(part 1 of 2)
# Autodesk Inventor assembly: mecanum_adaptive_trajectory
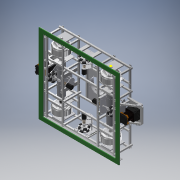
[picture p0: Inventor's stored thumbnail of the model, 180x180]
Saved by Autodesk Inventor 2018 (Build 220112000, 112)
## iProperties
Created: 2018-08-28
Part Number: mecanum_adaptive_trajectory
Material: 一般
Document SubType Name: Assembly
Designer: 澤田　将吾
Mass: 7709.16 g
Surface Area: 29088.3 cm^2
Volume: 5477.44 cm^3
Density: 1.40744 g/cm^3
Author: 澤田　将吾
## Documents named in this file (73)
- C:\Robohan\Svn\2018\自主研究\軌道追従2018\mecanum_adaptive_trajectory.iam
- C:\Robohan\Svn\2018\自主研究\軌道追従2018\既製品\14-KEY-RZ-735.ipt
- C:\Robohan\Svn\2018\自主研究\軌道追従2018\既製品\メカナムホイール.ipt
- C:\Robohan\Svn\2018\自主研究\軌道追従2018\parts\工場工作機\mecanum_wheel_shaft_holder.ipt
- C:\Robohan\Svn\2018\自主研究\軌道追従2018\既製品\mecanum_coupling.ipt
- C:\Robohan\Svn\2018\自主研究\軌道追従2018\parts\センター工作機\motor_plate.ipt
- C:\Robohan\Svn\2018\自主研究\軌道追従2018\parts\センターレーザー\motor-wheel_plate.ipt
- C:\Robohan\Svn\2018\自主研究\軌道追従2018\parts\センター工作機\mecanum_flameA.ipt
- C:\Robohan\Svn\2018\自主研究\軌道追従2018\parts\センター工作機\mecanum_flameB.ipt
- C:\Robohan\Svn\2018\自主研究\軌道追従2018\parts\工場工作機\mecanum_shaft.ipt
- C:\Robohan\Svn\2018\自主研究\軌道追従2018\既製品\14-KEY-RZ-736_MIR.ipt
- C:\Robohan\Svn\2018\自主研究\軌道追従2018\既製品\メカナムホイール_MIR.ipt
- C:\Robohan\Svn\2018\自主研究\軌道追従2018\parts\工場工作機\mecanum_wheel_shaft_holder_MIR.ipt
- C:\Robohan\Svn\2018\自主研究\軌道追従2018\既製品\mecanum_coupling_MIR.ipt
- C:\Robohan\Svn\2018\自主研究\軌道追従2018\parts\センター工作機\motor_plate_MIR.ipt
- C:\Robohan\Svn\2018\自主研究\軌道追従2018\parts\センターレーザー\motor-wheel_plate_MIR.ipt
- C:\Robohan\Svn\2018\自主研究\軌道追従2018\parts\センター工作機\mecanum_flameA_MIR.ipt
- C:\Robohan\Svn\2018\自主研究\軌道追従2018\parts\工場工作機\mecanum_shaft_MIR.ipt
- C:\Robohan\Svn\2018\自主研究\軌道追従2018\parts\センター工作機\mecanum_flameD.ipt
- C:\Robohan\Svn\2018\自主研究\軌道追従2018\parts\センター工作機\mecanum_flameE.ipt
- C:\Robohan\Svn\2018\自主研究\軌道追従2018\既製品\14-KEY-RZ-736_MIR1.ipt
- C:\Robohan\Svn\2018\自主研究\軌道追従2018\既製品\メカナムホイール_MIR1.ipt
- C:\Robohan\Svn\2018\自主研究\軌道追従2018\parts\工場工作機\mecanum_wheel_shaft_holder_MIR1.ipt
- C:\Robohan\Svn\2018\自主研究\軌道追従2018\既製品\mecanum_coupling_MIR1.ipt
- C:\Robohan\Svn\2018\自主研究\軌道追従2018\parts\センター工作機\motor_plate_MIR1.ipt
- C:\Robohan\Svn\2018\自主研究\軌道追従2018\parts\センターレーザー\motor-wheel_plate_MIR1.ipt
- C:\Robohan\Svn\2018\自主研究\軌道追従2018\parts\センター工作機\mecanum_flameA_MIR1.ipt
- C:\Robohan\Svn\2018\自主研究\軌道追従2018\parts\センター工作機\mecanum_flameB_MIR.ipt
- C:\Robohan\Svn\2018\自主研究\軌道追従2018\parts\工場工作機\mecanum_shaft_MIR1.ipt
- C:\Robohan\Svn\2018\自主研究\軌道追従2018\既製品\14-KEY-RZ-736_MIR_MIR.ipt
- C:\Robohan\Svn\2018\自主研究\軌道追従2018\既製品\メカナムホイール_MIR_MIR.ipt
- C:\Robohan\Svn\2018\自主研究\軌道追従2018\parts\工場工作機\mecanum_wheel_shaft_holder_MIR_MIR.ipt
- C:\Robohan\Svn\2018\自主研究\軌道追従2018\既製品\mecanum_coupling_MIR_MIR.ipt
- C:\Robohan\Svn\2018\自主研究\軌道追従2018\parts\センター工作機\motor_plate_MIR_MIR.ipt
- C:\Robohan\Svn\2018\自主研究\軌道追従2018\parts\センターレーザー\motor-wheel_plate_MIR_MIR.ipt
- C:\Robohan\Svn\2018\自主研究\軌道追従2018\parts\センター工作機\mecanum_flameA_MIR_MIR.ipt
- C:\Robohan\Svn\2018\自主研究\軌道追従2018\parts\工場工作機\mecanum_shaft_MIR_MIR.ipt
- C:\Robohan\Svn\2018\自主研究\軌道追従2018\parts\センター工作機\mecanum_flameE_MIR.ipt
- C:\Robohan\Svn\2018\自主研究\軌道追従2018\parts\センター工作機\mecanum_polycaplate.ipt
- C:\Robohan\Svn\2018\自主研究\軌道追従2018\parts\センター工作機\mecanum_polycaplateB.ipt
- C:\Robohan\Svn\2018\自主研究\軌道追従2018\parts\センター工作機\mecanum_polycaplateC.ipt
- C:\Robohan\Svn\2018\自主研究\軌道追従2018\parts\センター工作機\mecanum_angleA.ipt
- C:\Robohan\Svn\2018\自主研究\軌道追従2018\parts\センター工作機\mecanum_angleB.ipt
- C:\Robohan\Svn\2018\自主研究\軌道追従2018\既製品\fan_冶具-01.ipt
- C:\Robohan\Svn\2018\自主研究\軌道追従2018\既製品\bearingA.ipt
- C:\Robohan\Svn\2018\自主研究\軌道追従2018\既製品\mecanum_set_collarA.ipt
- C:\Robohan\Svn\2018\自主研究\軌道追従2018\既製品\Astuto_enc_wheel\Astuto_enc_wheel.iam
- C:\Robohan\Svn\2018\自主研究\軌道追従2018\parts\センター工作機\mecanum_encoder_shaftA.ipt
- C:\Robohan\Svn\2018\自主研究\軌道追従2018\parts\センターレーザー\mecanum_encoder_plateA.ipt
- C:\Robohan\Svn\2018\自主研究\軌道追従2018\parts\センターレーザー\mecanum_encoder_plateB.ipt
- C:\Robohan\Svn\2018\自主研究\軌道追従2018\parts\センター工作機\Astuto_enc_part1.ipt
- C:\Robohan\Svn\2018\自主研究\軌道追従2018\既製品\Astuto_enc_part2.ipt
- C:\Robohan\Svn\2018\自主研究\軌道追従2018\parts\センター工作機\mecanum_encoder_shaftB.ipt
- C:\Robohan\Svn\2018\自主研究\軌道追従2018\既製品\E6A2-CW3C.ipt
- C:\Robohan\Svn\2018\自主研究\軌道追従2018\parts\センターレーザー\mecanum_encoder_plateC.ipt
- C:\Robohan\Svn\2018\自主研究\軌道追従2018\parts\センター工作機\mecanum_encoder_shaftC.ipt
- C:\Robohan\Svn\2018\自主研究\軌道追従2018\parts\センター工作機\Astuto_enc_part3.ipt
- C:\Robohan\Svn\2018\自主研究\軌道追従2018\parts\センターレーザー\mecanum_encoder_plateD.ipt
- C:\Robohan\Svn\2018\自主研究\軌道追従2018\parts\センター工作機\mecanum_encoder_shaftD.ipt
- C:\Robohan\Svn\2018\自主研究\軌道追従2018\既製品\mecanum_encoder_coupling.ipt
- C:\Robohan\Svn\2018\自主研究\軌道追従2018\parts\センター工作機\mecanum_encoder_shaftE.ipt
- C:\Robohan\Svn\2018\自主研究\軌道追従2018\parts\センター工作機\mecanum_encoder_shaftF.ipt
- C:\Robohan\Svn\2018\自主研究\軌道追従2018\既製品\LRF\LRF.iam
- C:\Robohan\Svn\2018\自主研究\軌道追従2018\parts\センター工作機\mecanum_flameF.ipt
- C:\Robohan\Svn\2018\自主研究\軌道追従2018\parts\センター工作機\mecanum_LRF_flameA.ipt
- C:\Robohan\Svn\2018\自主研究\軌道追従2018\parts\センター工作機\mecanum_LRF_plate.ipt
- C:\Robohan\Svn\2018\自主研究\軌道追従2018\parts\センターレーザー\mecanum_gusset_plateA.ipt
- C:\Robohan\Svn\2018\自主研究\軌道追従2018\parts\センター工作機\mecanum_LRF_flameB.ipt
- C:\Robohan\Svn\2018\自主研究\軌道追従2018\parts\センター工作機\mecanum_kusaA.ipt
- C:\Robohan\Svn\2018\自主研究\軌道追従2018\parts\センター工作機\mecanum_kusaB.ipt
- C:\Robohan\Svn\2018\自主研究\軌道追従2018\parts\センター工作機\mecanum_flameG.ipt
- C:\Robohan\Svn\2018\自主研究\軌道追従2018\parts\センター工作機\mecanum_flameH.ipt
- C:\Robohan\Svn\2018\自主研究\軌道追従2018\parts\センターレーザー\mecanum_suction_motor_plate.ipt
## Components (196 placed, 73 different names)
1. 14-KEY-RZ-735:1 — メイト:1, メイト:2, 挿入:8, 挿入:9, 挿入:10, メイト:111
2. メカナムホイール:1 — 挿入:1, 挿入:2, 挿入:3
3. mecanum_wheel_shaft_holder:1 — 挿入:1, 挿入:2, 挿入:3, メイト:4, メイト:9, メイト:10
4. mecanum_coupling:1 — メイト:1, メイト:2, メイト:3, メイト:6, メイト:7, フラッシュ:1
5. motor_plate:1 — 挿入:8, 挿入:9, 挿入:10, メイト:7, 挿入:432, 挿入:433, 挿入:444, 挿入:445
6. motor-wheel_plate:1 — メイト:3, メイト:4, メイト:6, 挿入:4, 挿入:5, 挿入:31, 挿入:32, メイト:42
7. mecanum_flameA:1 — 挿入:4, 挿入:5, 挿入:6, 挿入:7
8. mecanum_flameB:1 — 挿入:6, 挿入:27, 挿入:30, 挿入:63, 挿入:65, 挿入:68, 挿入:71, 挿入:76, 挿入:81, 挿入:211, 挿入:214, 挿入:277, 挿入:278, 挿入:434, 挿入:472
9. mecanum_flameB:2 — 挿入:7, 挿入:28, 挿入:29, 挿入:49, 挿入:53, 挿入:57, 挿入:61, 挿入:75, 挿入:204, 挿入:206, 挿入:212, 挿入:213, 挿入:422, 挿入:424, 挿入:428, 挿入:429, 挿入:430, 挿入:476
10. mecanum_shaft:1 — メイト:9, フラッシュ:1, メイト:10, メイト:41, メイト:43, メイト:111
11. 14-KEY-RZ-736_MIR:1 — メイト:11, メイト:12, 挿入:18, 挿入:19, 挿入:20, メイト:112
12. メカナムホイール_MIR:1 — 挿入:15, 挿入:16, 挿入:17
13. mecanum_wheel_shaft_holder_MIR:1 — 挿入:15, 挿入:16, 挿入:17, メイト:16, メイト:18, メイト:20
14. mecanum_coupling_MIR:1 — メイト:11, メイト:12, メイト:13, メイト:14, メイト:17, メイト:19
15. motor_plate_MIR:1 — メイト:13, 挿入:18, 挿入:19, 挿入:20, 挿入:462, 挿入:463, 挿入:474, 挿入:475
16. motor-wheel_plate_MIR:1 — メイト:14, メイト:16, メイト:17, 挿入:21, 挿入:22, 挿入:40, 挿入:41, メイト:48
17. mecanum_flameA_MIR:1 — 挿入:21, 挿入:22, 挿入:27, 挿入:28
18. mecanum_shaft_MIR:1 — メイト:18, メイト:19, メイト:20, メイト:49, メイト:50, メイト:112
19. mecanum_flameD:1 — 挿入:29, 挿入:30, 挿入:54, 挿入:72, 挿入:153, 挿入:154, 挿入:158, 挿入:159, 挿入:185, 挿入:187, 挿入:190, 挿入:191, 挿入:194, 挿入:238, 挿入:239, 挿入:265, 挿入:266, 挿入:331, 挿入:334
20. mecanum_flameA:2 — 挿入:31, 挿入:32, 挿入:35, 挿入:43
21. mecanum_flameB:3 — 挿入:35, 挿入:42, 挿入:47, 挿入:52, 挿入:56, 挿入:60, 挿入:62, 挿入:78, メイト:67, 挿入:423, 挿入:425, 挿入:443, 挿入:447, 挿入:464, 挿入:465
22. mecanum_flameA_MIR:2 — 挿入:40, 挿入:41, 挿入:42, 挿入:46
23. mecanum_flameB:4 — 挿入:43, 挿入:46, 挿入:48, 挿入:64, 挿入:66, 挿入:69, 挿入:74, 挿入:80, 挿入:84, 挿入:275, 挿入:276, 挿入:446, 挿入:460
24. mecanum_flameD:2 — 挿入:47, 挿入:48, 挿入:55, 挿入:73, 挿入:155, 挿入:156, 挿入:157, 挿入:160, 挿入:186, 挿入:188, 挿入:189, 挿入:192, 挿入:193, 挿入:236, 挿入:237, 挿入:263, 挿入:264, 挿入:332, 挿入:333
25. mecanum_flameE:1 — 挿入:49, 挿入:52, 挿入:181, 挿入:182, 挿入:431, 挿入:442, 挿入:448
26. mecanum_flameE:2 — 挿入:53, 挿入:54, 挿入:55, 挿入:56, 挿入:183, 挿入:184
27. mecanum_flameE:3 — 挿入:57, 挿入:60, 挿入:179, 挿入:180, 挿入:465, 挿入:477
28. mecanum_flameE:4 — 挿入:61, 挿入:62, 挿入:77, 挿入:79, 挿入:177, 挿入:178
29. mecanum_flameE:5 — 挿入:63, 挿入:64, 挿入:68, 挿入:69, 挿入:435, 挿入:449
30. mecanum_flameE:6 — 挿入:65, 挿入:66, 挿入:461, 挿入:473
31. mecanum_flameE:7 — 挿入:71, 挿入:72, 挿入:73, 挿入:74
32. mecanum_flameD:3 — 挿入:75, 挿入:76, 挿入:77, 挿入:82, 挿入:161, 挿入:162, 挿入:165, 挿入:166, 挿入:195, 挿入:198, 挿入:199, 挿入:202, 挿入:249, 挿入:250, 挿入:267, 挿入:268, 挿入:296, 挿入:299
33. mecanum_flameD:4 — 挿入:78, 挿入:79, 挿入:80, 挿入:83, 挿入:163, 挿入:164, 挿入:167, 挿入:168, 挿入:196, 挿入:197, 挿入:200, 挿入:201, 挿入:247, 挿入:248, 挿入:269, 挿入:270, 挿入:297, 挿入:298
34. mecanum_flameE:8 — 挿入:81, 挿入:82, 挿入:83, 挿入:84
35. 14-KEY-RZ-736_MIR1:1 — メイト:22, メイト:23, 挿入:88, 挿入:89, 挿入:90, メイト:113
36. メカナムホイール_MIR1:1 — 挿入:85, 挿入:86, 挿入:87
37. mecanum_wheel_shaft_holder_MIR1:1 — 挿入:85, 挿入:86, 挿入:87, メイト:26, メイト:28, メイト:30
38. mecanum_coupling_MIR1:1 — メイト:22, メイト:23, メイト:24, メイト:25, メイト:27, メイト:29
39. motor_plate_MIR1:1 — メイト:24, 挿入:88, 挿入:89, 挿入:90, 挿入:438, 挿入:439, 挿入:452, 挿入:453
40. motor-wheel_plate_MIR1:1 — メイト:25, メイト:26, メイト:27, 挿入:91, 挿入:92, 挿入:113, 挿入:114, メイト:55
41. mecanum_flameA_MIR1:1 — 挿入:91, 挿入:92, 挿入:93, 挿入:94
42. mecanum_flameB_MIR:1 — 挿入:93, 挿入:106, 挿入:143, 挿入:146, 挿入:148, 挿入:150, 挿入:152, 挿入:153, 挿入:161, 挿入:208, 挿入:210, 挿入:350, 挿入:353, 挿入:437, 挿入:470
43. mecanum_flameB_MIR:2 — 挿入:94, 挿入:105, 挿入:132, 挿入:134, 挿入:138, 挿入:140, 挿入:159, 挿入:162, 挿入:203, 挿入:205, 挿入:207, 挿入:209, 挿入:372, 挿入:374, 挿入:426, 挿入:427, 挿入:440, 挿入:467
44. mecanum_shaft_MIR1:1 — メイト:28, メイト:29, メイト:30, メイト:56, メイト:57, メイト:113
45. 14-KEY-RZ-736_MIR_MIR:1 — メイト:32, メイト:33, 挿入:102, 挿入:103, 挿入:104, メイト:114
46. メカナムホイール_MIR_MIR:1 — 挿入:99, 挿入:100, 挿入:101
47. mecanum_wheel_shaft_holder_MIR_MIR:1 — 挿入:99, 挿入:100, 挿入:101, メイト:36, メイト:39, メイト:40
48. mecanum_coupling_MIR_MIR:1 — メイト:32, メイト:33, メイト:34, メイト:35, メイト:37, フラッシュ:2
49. motor_plate_MIR_MIR:1 — 挿入:102, 挿入:103, 挿入:104, メイト:34, 挿入:458, 挿入:468, 挿入:469
50. motor-wheel_plate_MIR_MIR:1 — メイト:35, メイト:36, メイト:37, 挿入:107, 挿入:108, 挿入:123, 挿入:124, メイト:58
51. mecanum_flameA_MIR_MIR:1 — 挿入:105, 挿入:106, 挿入:107, 挿入:108
52. mecanum_shaft_MIR_MIR:1 — メイト:39, フラッシュ:2, メイト:40, メイト:59, メイト:60, メイト:114
53. mecanum_flameA_MIR1:2 — 挿入:113, 挿入:114, 挿入:118, 挿入:128
54. mecanum_flameB_MIR:3 — 挿入:118, 挿入:122, 挿入:129, 挿入:133, 挿入:135, 挿入:139, 挿入:160, 挿入:164, 挿入:373, 挿入:375, 挿入:454, 挿入:457
55. mecanum_flameA_MIR_MIR:2 — 挿入:122, 挿入:123, 挿入:124, 挿入:125
56. mecanum_flameB_MIR:4 — 挿入:125, 挿入:128, 挿入:142, 挿入:145, 挿入:147, 挿入:149, 挿入:151, 挿入:155, 挿入:163, 挿入:351, 挿入:352, 挿入:450
57. mecanum_flameE_MIR:1 — 挿入:129, 挿入:132, 挿入:173, 挿入:174, 挿入:441, 挿入:455
58. mecanum_flameE_MIR:2 — 挿入:133, 挿入:134, 挿入:157, 挿入:158, 挿入:169, 挿入:170
59. mecanum_flameE_MIR:3 — 挿入:135, 挿入:138, 挿入:175, 挿入:176, 挿入:456, 挿入:466
60. mecanum_flameE_MIR:4 — 挿入:139, 挿入:140, 挿入:166, 挿入:167, 挿入:171, 挿入:172
61. mecanum_flameE_MIR:5 — 挿入:142, 挿入:143, 挿入:145, 挿入:146, 挿入:436, 挿入:451
62. mecanum_flameE_MIR:6 — 挿入:147, 挿入:148, 挿入:459, 挿入:471
63. mecanum_flameE_MIR:7 — 挿入:149, 挿入:150, 挿入:154, 挿入:156
64. mecanum_flameE_MIR:8 — 挿入:151, 挿入:152, 挿入:165, 挿入:168
65. mecanum_polycaplateA:1 — 挿入:169, 挿入:170, 挿入:171, 挿入:172, 挿入:173, 挿入:174, 挿入:175, 挿入:176, 挿入:215, 挿入:216, 挿入:217, 挿入:218
66. mecanum_polycaplate:2 — 挿入:177, 挿入:178, 挿入:179, 挿入:180, 挿入:181, 挿入:182, 挿入:183, 挿入:184, 挿入:219, 挿入:220, 挿入:221, 挿入:222
67. mecanum_polycaplateB:1 — 挿入:185, 挿入:186, 挿入:187, 挿入:188, 挿入:189, 挿入:190, 挿入:191, 挿入:192, 挿入:193, 挿入:194, 挿入:223, 挿入:224, 挿入:225, 挿入:226
68. mecanum_polycaplateB:2 — 挿入:195, 挿入:196, 挿入:197, 挿入:198, 挿入:199, 挿入:200, 挿入:201, 挿入:202, 挿入:227, 挿入:228, 挿入:229, 挿入:230
69. mecanum_polycaplateC:1 — 挿入:203, 挿入:204, 挿入:205, 挿入:206, 挿入:207, 挿入:208, 挿入:209, 挿入:210, 挿入:211, 挿入:212, 挿入:213, 挿入:214
70. mecanum_angleA:1 — 挿入:215, 挿入:216, 挿入:217, 挿入:218, フラッシュ:15, フラッシュ:16, メイト:108
71. mecanum_angleA:2 — 挿入:219, 挿入:220, 挿入:221, 挿入:222, メイト:107, フラッシュ:13, フラッシュ:14
72. mecanum_angleB:1 — 挿入:223, 挿入:224, 挿入:225, 挿入:226, フラッシュ:19, フラッシュ:20, メイト:110
73. mecanum_angleB:2 — 挿入:227, 挿入:228, 挿入:229, 挿入:230, メイト:109, フラッシュ:17, フラッシュ:18
74. fan_冶具-01:1 — 挿入:486, 挿入:487, 挿入:488, 挿入:489, 挿入:490
75. bearingA:1 — メイト:41, メイト:42, 挿入:231
76. mecanum_set_collarA:1 — 挿入:231
77. motor-wheel_plate:2 — メイト:43, 挿入:232, 挿入:233, 挿入:234, 挿入:235, メイト:44, メイト:45
78. motor-wheel_plate:3 — 挿入:232, 挿入:233, 挿入:234, 挿入:235, 挿入:236, 挿入:237, 挿入:238, 挿入:239
79. bearingA:2 — メイト:44, メイト:45, 挿入:240
80. mecanum_set_collarA:2 — 挿入:240
81. bearingA:3 — メイト:48, メイト:49
82. mecanum_set_collarA:3
83. motor-wheel_plate:4
84. motor-wheel_plate:5 — 挿入:247, 挿入:248, 挿入:249, 挿入:250
85. bearingA:4 — メイト:50
86. mecanum_set_collarA:4
87. bearingA:5 — メイト:55
88. mecanum_set_collarA:5 — メイト:56
89. motor-wheel_plate:6
90. motor-wheel_plate:7 — 挿入:263, 挿入:264, 挿入:265, 挿入:266
91. bearingA:6 — メイト:57
92. mecanum_set_collarA:6
93. bearingA:7 — メイト:58, メイト:59
94. mecanum_set_collarA:7
95. motor-wheel_plate:8
96. motor-wheel_plate:9 — 挿入:267, 挿入:268, 挿入:269, 挿入:270
97. bearingA:8 — メイト:60
98. mecanum_set_collarA:8
99. Astuto_enc_wheel:1 [sub-assembly] — メイト:61, メイト:91
100. mecanum_encoder_shaftA:1 — メイト:61, メイト:62, メイト:68, メイト:69, フラッシュ:4, メイト:77
101. mecanum_encoder_plateA:1 — メイト:67, メイト:68, 挿入:281, 挿入:282, フラッシュ:4, メイト:91
102. mecanum_encoder_plateB:1 — メイト:62, 挿入:271, 挿入:272, 挿入:273, 挿入:274, 挿入:280, メイト:70, 挿入:288, 挿入:289, 挿入:290
103. Astuto_enc_part1:2 — メイト:63, メイト:64, 挿入:275, 挿入:278, フラッシュ:3
104. Astuto_enc_part2:2 — メイト:63, メイト:64, 挿入:271, 挿入:272, フラッシュ:3
105. Astuto_enc_part1:3 — 挿入:276, 挿入:277, メイト:66
106. Astuto_enc_part2:3 — 挿入:273, 挿入:274, メイト:66
107. mecanum_encoder_shaftB:1 — 挿入:280, 挿入:281
108. mecanum_encoder_shaftB:2 — 挿入:282
109. E6A2-CW3C:1 — 挿入:283, 挿入:284, メイト:69
110. mecanum_encoder_plateC:1 — 挿入:283, 挿入:284, 挿入:285, 挿入:286, 挿入:287, メイト:78
111. mecanum_encoder_shaftC:1 — 挿入:285, メイト:70, 挿入:289
112. mecanum_encoder_shaftC:2 — 挿入:287, 挿入:290
113. mecanum_encoder_shaftC:3 — 挿入:286, 挿入:288
114. Astuto_enc_wheel:2 [sub-assembly] — メイト:76, メイト:79, メイト:81, メイト:105
115. E6A2-CW3C:2
116. mecanum_encoder_plateC:2 — メイト:80, 挿入:361, 挿入:362, 挿入:363
117. Astuto_enc_part3:1 — 挿入:296, 挿入:297, メイト:72, メイト:74
118. Astuto_enc_part3:2 — 挿入:298, 挿入:299, メイト:73, メイト:75, フラッシュ:6
119. Astuto_enc_part2:4 — メイト:73, メイト:75, 挿入:300, 挿入:303, フラッシュ:6
120. Astuto_enc_part2:5 — メイト:72, メイト:74, 挿入:301, 挿入:302
121. mecanum_encoder_plateD:1 — 挿入:300, 挿入:301, 挿入:302, 挿入:303, メイト:76, 挿入:304, 挿入:305, 挿入:306, フラッシュ:7, メイト:105
122. mecanum_encoder_shaftD:1 — 挿入:304, 挿入:307
123. mecanum_encoder_shaftD:2 — 挿入:305, 挿入:308
124. mecanum_encoder_shaftD:3 — 挿入:306, 挿入:309
125. mecanum_encoder_plateC:3 — 挿入:307, 挿入:308, 挿入:309, 挿入:360, 挿入:364, 挿入:365
126. mecanum_encoder_coupling:1 — メイト:77, メイト:78
127. mecanum_encoder_coupling:2 — メイト:79, メイト:80
128. mecanum_encoder_shaftE:1 — メイト:81, フラッシュ:7
129. Astuto_enc_wheel:3 [sub-assembly] — メイト:106
130. E6A2-CW3C:3
131. mecanum_encoder_plateC:4 — 挿入:355, 挿入:356, 挿入:357
132. Astuto_enc_part3:3 — 挿入:331, 挿入:332
133. Astuto_enc_part3:4 — 挿入:333, 挿入:334
134. Astuto_enc_part2:6
135. Astuto_enc_part2:7
136. mecanum_encoder_plateD:2 — メイト:106
137. mecanum_encoder_shaftD:4
138. mecanum_encoder_shaftD:5
139. mecanum_encoder_shaftD:6
140. mecanum_encoder_plateC:5 — 挿入:354, 挿入:358, 挿入:359
141. mecanum_encoder_coupling:3
142. mecanum_encoder_shaftE:2
143. Astuto_enc_wheel:4 [sub-assembly]
144. mecanum_encoder_shaftA:2
145. mecanum_encoder_plateA:2
146. mecanum_encoder_plateB:2
147. Astuto_enc_part1:4 — 挿入:350, 挿入:351
148. Astuto_enc_part2:8
149. Astuto_enc_part1:5 — 挿入:352, 挿入:353
150. Astuto_enc_part2:9
151. mecanum_encoder_shaftB:3
152. mecanum_encoder_shaftB:4
153. E6A2-CW3C:4
154. mecanum_encoder_plateC:6
155. mecanum_encoder_shaftC:10
156. mecanum_encoder_shaftC:11
157. mecanum_encoder_shaftC:12
158. mecanum_encoder_coupling:4
159. mecanum_encoder_shaftF:1 — 挿入:354, 挿入:355
160. mecanum_encoder_shaftF:2 — 挿入:356, 挿入:358
161. mecanum_encoder_shaftF:3 — 挿入:357, 挿入:359
162. mecanum_encoder_shaftF:4 — 挿入:360, 挿入:361
163. mecanum_encoder_shaftF:5 — 挿入:362, 挿入:364
164. mecanum_encoder_shaftF:6 — 挿入:363, 挿入:365
165. fan_冶具-01:2 — 挿入:491, 挿入:492, 挿入:493, 挿入:494
166. LRF:1 [sub-assembly] — 挿入:384, 挿入:385, 挿入:386, 挿入:387
167. mecanum_flameF:1 — 挿入:372, 挿入:373, 挿入:377, 挿入:394
168. mecanum_flameF:2 — 挿入:374, 挿入:375, 挿入:379, 挿入:401
169. mecanum_LRF_flameA:1 — 挿入:377, 挿入:388, 挿入:389, 挿入:392, 挿入:393, 挿入:427
170. mecanum_LRF_flameA:2 — 挿入:379, 挿入:390, 挿入:391, 挿入:397, 挿入:398, 挿入:426
171. mecanum_LRF_plate:1 — 挿入:384, 挿入:385, 挿入:386, 挿入:387, 挿入:388, 挿入:389, 挿入:390, 挿入:391
172. mecanum_gusset_plateA:1 — 挿入:392, 挿入:393, 挿入:395, 挿入:396
173. mecanum_LRF_flameB:1 — 挿入:394, 挿入:395, 挿入:396
174. mecanum_gusset_plateA:2 — 挿入:397, 挿入:398, 挿入:399, 挿入:400
175. mecanum_LRF_flameB:2 — 挿入:399, 挿入:400, 挿入:401
176. LRF:3 [sub-assembly]
177. mecanum_flameF:3 — 挿入:422, 挿入:423
178. mecanum_flameF:4 — 挿入:424, 挿入:425
179. mecanum_LRF_flameA:3 — 挿入:428
180. mecanum_LRF_flameA:4 — 挿入:429
181. mecanum_LRF_plate:2
182. mecanum_gusset_plateA:3
183. mecanum_LRF_flameB:3
184. mecanum_gusset_plateA:4
185. mecanum_LRF_flameB:4
186. mecanum_kusaA:1 — フラッシュ:15, フラッシュ:16, メイト:108
187. mecanum_kusaA:2 — メイト:107, フラッシュ:13, フラッシュ:14
188. mecanum_kusaB:1 — メイト:109, フラッシュ:17, フラッシュ:18
189. mecanum_kusaB:2 — フラッシュ:19, フラッシュ:20, メイト:110
190. mecanum_flameG:1 — 挿入:430, 挿入:431, 挿入:432, 挿入:433, 挿入:434, 挿入:435, 挿入:436, 挿入:437, 挿入:438, 挿入:439, 挿入:440, 挿入:441, 挿入:479, 挿入:481
191. mecanum_flameG:2 — 挿入:442, 挿入:443, 挿入:444, 挿入:445, 挿入:446, 挿入:447, 挿入:448, 挿入:449, 挿入:450, 挿入:451, 挿入:452, 挿入:453, 挿入:454, 挿入:455
192. mecanum_flameG:3 — 挿入:456, 挿入:457, 挿入:458, 挿入:459, 挿入:460, 挿入:461, 挿入:462, 挿入:463, 挿入:464
193. mecanum_flameG:4 — 挿入:466, 挿入:467, 挿入:468, 挿入:469, 挿入:470, 挿入:471, 挿入:472, 挿入:473, 挿入:474, 挿入:475, 挿入:476, 挿入:477, 挿入:478, 挿入:480
194. mecanum_flameH:1 — 挿入:478, 挿入:479, 挿入:482, 挿入:484
195. mecanum_suction_motor_plate:1 — 挿入:482, 挿入:483, 挿入:484, 挿入:485, 挿入:486, 挿入:487, 挿入:488, 挿入:489, 挿入:490, 挿入:491, 挿入:492, 挿入:493, 挿入:494
196. mecanum_flameH:2 — 挿入:480, 挿入:481, 挿入:483, 挿入:485
## Relationships (548: Insert 425, Mate 105, Flush 18)
- 挿入:1 [Insert]: メカナムホイール:1 ↔ mecanum_wheel_shaft_holder:1
- 挿入:2 [Insert]: メカナムホイール:1 ↔ mecanum_wheel_shaft_holder:1
- 挿入:3 [Insert]: メカナムホイール:1 ↔ mecanum_wheel_shaft_holder:1
- メイト:1 [Mate]: 14-KEY-RZ-735:1 ↔ mecanum_coupling:1
- メイト:2 [Mate] (3 mm): 14-KEY-RZ-735:1 ↔ mecanum_coupling:1
- メイト:3 [Mate]: mecanum_coupling:1 ↔ motor-wheel_plate:1
- メイト:4 [Mate]: mecanum_wheel_shaft_holder:1 ↔ motor-wheel_plate:1
- メイト:6 [Mate] (5 mm): mecanum_coupling:1 ↔ motor-wheel_plate:1
- 挿入:4 [Insert]: motor-wheel_plate:1 ↔ mecanum_flameA:1
- 挿入:5 [Insert]: motor-wheel_plate:1 ↔ mecanum_flameA:1
- 挿入:6 [Insert]: mecanum_flameA:1 ↔ mecanum_flameB:1
- 挿入:7 [Insert]: mecanum_flameA:1 ↔ mecanum_flameB:2
- 挿入:8 [Insert]: 14-KEY-RZ-735:1 ↔ motor_plate:1
- 挿入:9 [Insert]: 14-KEY-RZ-735:1 ↔ motor_plate:1
- 挿入:10 [Insert]: 14-KEY-RZ-735:1 ↔ motor_plate:1
- メイト:7 [Mate] (5 mm): mecanum_coupling:1 ↔ motor_plate:1
- メイト:9 [Mate]: mecanum_wheel_shaft_holder:1 ↔ mecanum_shaft:1
- フラッシュ:1 [Flush]: mecanum_coupling:1 ↔ mecanum_shaft:1
- メイト:10 [Mate]: mecanum_wheel_shaft_holder:1 ↔ mecanum_shaft:1
- 挿入:15 [Insert]: メカナムホイール_MIR:1 ↔ mecanum_wheel_shaft_holder_MIR:1
- 挿入:16 [Insert]: メカナムホイール_MIR:1 ↔ mecanum_wheel_shaft_holder_MIR:1
- 挿入:17 [Insert]: メカナムホイール_MIR:1 ↔ mecanum_wheel_shaft_holder_MIR:1
- メイト:11 [Mate] (3 mm): 14-KEY-RZ-736_MIR:1 ↔ mecanum_coupling_MIR:1
- メイト:12 [Mate]: 14-KEY-RZ-736_MIR:1 ↔ mecanum_coupling_MIR:1
- メイト:13 [Mate] (5 mm): mecanum_coupling_MIR:1 ↔ motor_plate_MIR:1
- 挿入:18 [Insert]: 14-KEY-RZ-736_MIR:1 ↔ motor_plate_MIR:1
- 挿入:19 [Insert]: 14-KEY-RZ-736_MIR:1 ↔ motor_plate_MIR:1
- 挿入:20 [Insert]: 14-KEY-RZ-736_MIR:1 ↔ motor_plate_MIR:1
- メイト:14 [Mate] (5 mm): mecanum_coupling_MIR:1 ↔ motor-wheel_plate_MIR:1
- メイト:16 [Mate]: mecanum_wheel_shaft_holder_MIR:1 ↔ motor-wheel_plate_MIR:1
- メイト:17 [Mate]: mecanum_coupling_MIR:1 ↔ motor-wheel_plate_MIR:1
- 挿入:21 [Insert]: motor-wheel_plate_MIR:1 ↔ mecanum_flameA_MIR:1
- 挿入:22 [Insert]: motor-wheel_plate_MIR:1 ↔ mecanum_flameA_MIR:1
- メイト:18 [Mate]: mecanum_wheel_shaft_holder_MIR:1 ↔ mecanum_shaft_MIR:1
- メイト:19 [Mate]: mecanum_coupling_MIR:1 ↔ mecanum_shaft_MIR:1
- メイト:20 [Mate]: mecanum_wheel_shaft_holder_MIR:1 ↔ mecanum_shaft_MIR:1
- 挿入:27 [Insert]: mecanum_flameB:1 ↔ mecanum_flameA_MIR:1
- 挿入:28 [Insert]: mecanum_flameB:2 ↔ mecanum_flameA_MIR:1
- 挿入:29 [Insert]: mecanum_flameB:2 ↔ mecanum_flameD:1
- 挿入:30 [Insert]: mecanum_flameB:1 ↔ mecanum_flameD:1
- 挿入:31 [Insert]: motor-wheel_plate:1 ↔ mecanum_flameA:2
- 挿入:32 [Insert]: motor-wheel_plate:1 ↔ mecanum_flameA:2
- 挿入:35 [Insert]: mecanum_flameA:2 ↔ mecanum_flameB:3
- 挿入:40 [Insert]: motor-wheel_plate_MIR:1 ↔ mecanum_flameA_MIR:2
- 挿入:41 [Insert]: motor-wheel_plate_MIR:1 ↔ mecanum_flameA_MIR:2
- 挿入:42 [Insert]: mecanum_flameB:3 ↔ mecanum_flameA_MIR:2
- 挿入:43 [Insert]: mecanum_flameA:2 ↔ mecanum_flameB:4
- 挿入:46 [Insert]: mecanum_flameA_MIR:2 ↔ mecanum_flameB:4
- 挿入:47 [Insert]: mecanum_flameB:3 ↔ mecanum_flameD:2
- 挿入:48 [Insert]: mecanum_flameB:4 ↔ mecanum_flameD:2
- 挿入:49 [Insert]: mecanum_flameB:2 ↔ mecanum_flameE:1
- 挿入:52 [Insert]: mecanum_flameB:3 ↔ mecanum_flameE:1
- 挿入:53 [Insert]: mecanum_flameB:2 ↔ mecanum_flameE:2
- 挿入:54 [Insert]: mecanum_flameD:1 ↔ mecanum_flameE:2
- 挿入:55 [Insert]: mecanum_flameD:2 ↔ mecanum_flameE:2
- 挿入:56 [Insert]: mecanum_flameB:3 ↔ mecanum_flameE:2
- 挿入:57 [Insert]: mecanum_flameB:2 ↔ mecanum_flameE:3
- 挿入:60 [Insert]: mecanum_flameB:3 ↔ mecanum_flameE:3
- 挿入:61 [Insert]: mecanum_flameB:2 ↔ mecanum_flameE:4
- 挿入:62 [Insert]: mecanum_flameB:3 ↔ mecanum_flameE:4
- 挿入:63 [Insert]: mecanum_flameB:1 ↔ mecanum_flameE:5
- 挿入:64 [Insert]: mecanum_flameB:4 ↔ mecanum_flameE:5
- 挿入:65 [Insert]: mecanum_flameB:1 ↔ mecanum_flameE:6
- 挿入:66 [Insert]: mecanum_flameB:4 ↔ mecanum_flameE:6
- 挿入:68 [Insert]: mecanum_flameB:1 ↔ mecanum_flameE:5
- 挿入:69 [Insert]: mecanum_flameB:4 ↔ mecanum_flameE:5
- 挿入:71 [Insert]: mecanum_flameB:1 ↔ mecanum_flameE:7
- 挿入:72 [Insert]: mecanum_flameD:1 ↔ mecanum_flameE:7
- 挿入:73 [Insert]: mecanum_flameD:2 ↔ mecanum_flameE:7
- 挿入:74 [Insert]: mecanum_flameB:4 ↔ mecanum_flameE:7
- 挿入:75 [Insert]: mecanum_flameB:2 ↔ mecanum_flameD:3
- 挿入:76 [Insert]: mecanum_flameB:1 ↔ mecanum_flameD:3
- 挿入:77 [Insert]: mecanum_flameE:4 ↔ mecanum_flameD:3
- 挿入:78 [Insert]: mecanum_flameB:3 ↔ mecanum_flameD:4
- 挿入:79 [Insert]: mecanum_flameE:4 ↔ mecanum_flameD:4
- 挿入:80 [Insert]: mecanum_flameB:4 ↔ mecanum_flameD:4
- 挿入:81 [Insert]: mecanum_flameB:1 ↔ mecanum_flameE:8
- 挿入:82 [Insert]: mecanum_flameD:3 ↔ mecanum_flameE:8
- 挿入:83 [Insert]: mecanum_flameD:4 ↔ mecanum_flameE:8
- 挿入:84 [Insert]: mecanum_flameB:4 ↔ mecanum_flameE:8
- 挿入:85 [Insert]: メカナムホイール_MIR1:1 ↔ mecanum_wheel_shaft_holder_MIR1:1
- 挿入:86 [Insert]: メカナムホイール_MIR1:1 ↔ mecanum_wheel_shaft_holder_MIR1:1
- 挿入:87 [Insert]: メカナムホイール_MIR1:1 ↔ mecanum_wheel_shaft_holder_MIR1:1
- メイト:22 [Mate] (3 mm): 14-KEY-RZ-736_MIR1:1 ↔ mecanum_coupling_MIR1:1
- メイト:23 [Mate]: 14-KEY-RZ-736_MIR1:1 ↔ mecanum_coupling_MIR1:1
- メイト:24 [Mate] (5 mm): mecanum_coupling_MIR1:1 ↔ motor_plate_MIR1:1
- 挿入:88 [Insert]: 14-KEY-RZ-736_MIR1:1 ↔ motor_plate_MIR1:1
- 挿入:89 [Insert]: 14-KEY-RZ-736_MIR1:1 ↔ motor_plate_MIR1:1
- 挿入:90 [Insert]: 14-KEY-RZ-736_MIR1:1 ↔ motor_plate_MIR1:1
- メイト:25 [Mate] (5 mm): mecanum_coupling_MIR1:1 ↔ motor-wheel_plate_MIR1:1
- メイト:26 [Mate]: mecanum_wheel_shaft_holder_MIR1:1 ↔ motor-wheel_plate_MIR1:1
- メイト:27 [Mate]: mecanum_coupling_MIR1:1 ↔ motor-wheel_plate_MIR1:1
- 挿入:91 [Insert]: motor-wheel_plate_MIR1:1 ↔ mecanum_flameA_MIR1:1
- 挿入:92 [Insert]: motor-wheel_plate_MIR1:1 ↔ mecanum_flameA_MIR1:1
- 挿入:93 [Insert]: mecanum_flameA_MIR1:1 ↔ mecanum_flameB_MIR:1
- 挿入:94 [Insert]: mecanum_flameA_MIR1:1 ↔ mecanum_flameB_MIR:2
- メイト:28 [Mate]: mecanum_wheel_shaft_holder_MIR1:1 ↔ mecanum_shaft_MIR1:1
- メイト:29 [Mate]: mecanum_coupling_MIR1:1 ↔ mecanum_shaft_MIR1:1
- メイト:30 [Mate]: mecanum_wheel_shaft_holder_MIR1:1 ↔ mecanum_shaft_MIR1:1
- 挿入:99 [Insert]: メカナムホイール_MIR_MIR:1 ↔ mecanum_wheel_shaft_holder_MIR_MIR:1
- 挿入:100 [Insert]: メカナムホイール_MIR_MIR:1 ↔ mecanum_wheel_shaft_holder_MIR_MIR:1
- 挿入:101 [Insert]: メカナムホイール_MIR_MIR:1 ↔ mecanum_wheel_shaft_holder_MIR_MIR:1
- メイト:32 [Mate]: 14-KEY-RZ-736_MIR_MIR:1 ↔ mecanum_coupling_MIR_MIR:1
- メイト:33 [Mate] (3 mm): 14-KEY-RZ-736_MIR_MIR:1 ↔ mecanum_coupling_MIR_MIR:1
- 挿入:102 [Insert]: 14-KEY-RZ-736_MIR_MIR:1 ↔ motor_plate_MIR_MIR:1
- 挿入:103 [Insert]: 14-KEY-RZ-736_MIR_MIR:1 ↔ motor_plate_MIR_MIR:1
- 挿入:104 [Insert]: 14-KEY-RZ-736_MIR_MIR:1 ↔ motor_plate_MIR_MIR:1
- メイト:34 [Mate] (5 mm): mecanum_coupling_MIR_MIR:1 ↔ motor_plate_MIR_MIR:1
- メイト:35 [Mate]: mecanum_coupling_MIR_MIR:1 ↔ motor-wheel_plate_MIR_MIR:1
- メイト:36 [Mate]: mecanum_wheel_shaft_holder_MIR_MIR:1 ↔ motor-wheel_plate_MIR_MIR:1
- メイト:37 [Mate] (5 mm): mecanum_coupling_MIR_MIR:1 ↔ motor-wheel_plate_MIR_MIR:1
- 挿入:105 [Insert]: mecanum_flameB_MIR:2 ↔ mecanum_flameA_MIR_MIR:1
- 挿入:106 [Insert]: mecanum_flameB_MIR:1 ↔ mecanum_flameA_MIR_MIR:1
- 挿入:107 [Insert]: motor-wheel_plate_MIR_MIR:1 ↔ mecanum_flameA_MIR_MIR:1
- 挿入:108 [Insert]: motor-wheel_plate_MIR_MIR:1 ↔ mecanum_flameA_MIR_MIR:1
- メイト:39 [Mate]: mecanum_wheel_shaft_holder_MIR_MIR:1 ↔ mecanum_shaft_MIR_MIR:1
- フラッシュ:2 [Flush]: mecanum_coupling_MIR_MIR:1 ↔ mecanum_shaft_MIR_MIR:1
- メイト:40 [Mate]: mecanum_wheel_shaft_holder_MIR_MIR:1 ↔ mecanum_shaft_MIR_MIR:1
- 挿入:113 [Insert]: motor-wheel_plate_MIR1:1 ↔ mecanum_flameA_MIR1:2
- 挿入:114 [Insert]: motor-wheel_plate_MIR1:1 ↔ mecanum_flameA_MIR1:2
- 挿入:118 [Insert]: mecanum_flameA_MIR1:2 ↔ mecanum_flameB_MIR:3
- 挿入:122 [Insert]: mecanum_flameB_MIR:3 ↔ mecanum_flameA_MIR_MIR:2
- 挿入:123 [Insert]: motor-wheel_plate_MIR_MIR:1 ↔ mecanum_flameA_MIR_MIR:2
- 挿入:124 [Insert]: motor-wheel_plate_MIR_MIR:1 ↔ mecanum_flameA_MIR_MIR:2
- 挿入:125 [Insert]: mecanum_flameA_MIR_MIR:2 ↔ mecanum_flameB_MIR:4
- 挿入:128 [Insert]: mecanum_flameA_MIR1:2 ↔ mecanum_flameB_MIR:4
- 挿入:129 [Insert]: mecanum_flameB_MIR:3 ↔ mecanum_flameE_MIR:1
- 挿入:132 [Insert]: mecanum_flameB_MIR:2 ↔ mecanum_flameE_MIR:1
- 挿入:133 [Insert]: mecanum_flameB_MIR:3 ↔ mecanum_flameE_MIR:2
- 挿入:134 [Insert]: mecanum_flameB_MIR:2 ↔ mecanum_flameE_MIR:2
- 挿入:135 [Insert]: mecanum_flameB_MIR:3 ↔ mecanum_flameE_MIR:3
- 挿入:138 [Insert]: mecanum_flameB_MIR:2 ↔ mecanum_flameE_MIR:3
- 挿入:139 [Insert]: mecanum_flameB_MIR:3 ↔ mecanum_flameE_MIR:4
- 挿入:140 [Insert]: mecanum_flameB_MIR:2 ↔ mecanum_flameE_MIR:4
- 挿入:142 [Insert]: mecanum_flameB_MIR:4 ↔ mecanum_flameE_MIR:5
- 挿入:143 [Insert]: mecanum_flameB_MIR:1 ↔ mecanum_flameE_MIR:5
- 挿入:145 [Insert]: mecanum_flameB_MIR:4 ↔ mecanum_flameE_MIR:5
- 挿入:146 [Insert]: mecanum_flameB_MIR:1 ↔ mecanum_flameE_MIR:5
- 挿入:147 [Insert]: mecanum_flameB_MIR:4 ↔ mecanum_flameE_MIR:6
- 挿入:148 [Insert]: mecanum_flameB_MIR:1 ↔ mecanum_flameE_MIR:6
- 挿入:149 [Insert]: mecanum_flameB_MIR:4 ↔ mecanum_flameE_MIR:7
- 挿入:150 [Insert]: mecanum_flameB_MIR:1 ↔ mecanum_flameE_MIR:7
- 挿入:151 [Insert]: mecanum_flameB_MIR:4 ↔ mecanum_flameE_MIR:8
- 挿入:152 [Insert]: mecanum_flameB_MIR:1 ↔ mecanum_flameE_MIR:8
- 挿入:153 [Insert]: mecanum_flameD:1 ↔ mecanum_flameB_MIR:1
- 挿入:154 [Insert]: mecanum_flameD:1 ↔ mecanum_flameE_MIR:7
- 挿入:155 [Insert]: mecanum_flameD:2 ↔ mecanum_flameB_MIR:4
- 挿入:156 [Insert]: mecanum_flameD:2 ↔ mecanum_flameE_MIR:7
- 挿入:157 [Insert]: mecanum_flameD:2 ↔ mecanum_flameE_MIR:2
- 挿入:158 [Insert]: mecanum_flameD:1 ↔ mecanum_flameE_MIR:2
- 挿入:159 [Insert]: mecanum_flameD:1 ↔ mecanum_flameB_MIR:2
- 挿入:160 [Insert]: mecanum_flameD:2 ↔ mecanum_flameB_MIR:3
- 挿入:161 [Insert]: mecanum_flameD:3 ↔ mecanum_flameB_MIR:1
- 挿入:162 [Insert]: mecanum_flameD:3 ↔ mecanum_flameB_MIR:2
- 挿入:163 [Insert]: mecanum_flameD:4 ↔ mecanum_flameB_MIR:4
- 挿入:164 [Insert]: mecanum_flameD:4 ↔ mecanum_flameB_MIR:3
- 挿入:165 [Insert]: mecanum_flameD:3 ↔ mecanum_flameE_MIR:8
- 挿入:166 [Insert]: mecanum_flameD:3 ↔ mecanum_flameE_MIR:4
- 挿入:167 [Insert]: mecanum_flameD:4 ↔ mecanum_flameE_MIR:4
- 挿入:168 [Insert]: mecanum_flameD:4 ↔ mecanum_flameE_MIR:8
- 挿入:169 [Insert]: mecanum_flameE_MIR:2 ↔ mecanum_polycaplateA:1
- 挿入:170 [Insert]: mecanum_flameE_MIR:2 ↔ mecanum_polycaplateA:1
- 挿入:171 [Insert]: mecanum_flameE_MIR:4 ↔ mecanum_polycaplateA:1
- 挿入:172 [Insert]: mecanum_flameE_MIR:4 ↔ mecanum_polycaplateA:1
- 挿入:173 [Insert]: mecanum_flameE_MIR:1 ↔ mecanum_polycaplateA:1
- 挿入:174 [Insert]: mecanum_flameE_MIR:1 ↔ mecanum_polycaplateA:1
- 挿入:175 [Insert]: mecanum_flameE_MIR:3 ↔ mecanum_polycaplateA:1
- 挿入:176 [Insert]: mecanum_flameE_MIR:3 ↔ mecanum_polycaplateA:1
- 挿入:177 [Insert]: mecanum_flameE:4 ↔ mecanum_polycaplate:2
- 挿入:178 [Insert]: mecanum_flameE:4 ↔ mecanum_polycaplate:2
- 挿入:179 [Insert]: mecanum_flameE:3 ↔ mecanum_polycaplate:2
- 挿入:180 [Insert]: mecanum_flameE:3 ↔ mecanum_polycaplate:2
- 挿入:181 [Insert]: mecanum_flameE:1 ↔ mecanum_polycaplate:2
- 挿入:182 [Insert]: mecanum_flameE:1 ↔ mecanum_polycaplate:2
- 挿入:183 [Insert]: mecanum_flameE:2 ↔ mecanum_polycaplate:2
- 挿入:184 [Insert]: mecanum_flameE:2 ↔ mecanum_polycaplate:2
- 挿入:185 [Insert]: mecanum_flameD:1 ↔ mecanum_polycaplateB:1
- 挿入:186 [Insert]: mecanum_flameD:2 ↔ mecanum_polycaplateB:1
- 挿入:187 [Insert]: mecanum_flameD:1 ↔ mecanum_polycaplateB:1
- 挿入:188 [Insert]: mecanum_flameD:2 ↔ mecanum_polycaplateB:1
- 挿入:189 [Insert]: mecanum_flameD:2 ↔ mecanum_polycaplateB:1
- 挿入:190 [Insert]: mecanum_flameD:1 ↔ mecanum_polycaplateB:1
- 挿入:191 [Insert]: mecanum_flameD:1 ↔ mecanum_polycaplateB:1
- 挿入:192 [Insert]: mecanum_flameD:2 ↔ mecanum_polycaplateB:1
- 挿入:193 [Insert]: mecanum_flameD:2 ↔ mecanum_polycaplateB:1
- 挿入:194 [Insert]: mecanum_flameD:1 ↔ mecanum_polycaplateB:1
- 挿入:195 [Insert]: mecanum_flameD:3 ↔ mecanum_polycaplateB:2
- 挿入:196 [Insert]: mecanum_flameD:4 ↔ mecanum_polycaplateB:2
- 挿入:197 [Insert]: mecanum_flameD:4 ↔ mecanum_polycaplateB:2
- 挿入:198 [Insert]: mecanum_flameD:3 ↔ mecanum_polycaplateB:2
- 挿入:199 [Insert]: mecanum_flameD:3 ↔ mecanum_polycaplateB:2
- 挿入:200 [Insert]: mecanum_flameD:4 ↔ mecanum_polycaplateB:2
- 挿入:201 [Insert]: mecanum_flameD:4 ↔ mecanum_polycaplateB:2
- 挿入:202 [Insert]: mecanum_flameD:3 ↔ mecanum_polycaplateB:2
- 挿入:203 [Insert]: mecanum_flameB_MIR:2 ↔ mecanum_polycaplateC:1
- 挿入:204 [Insert]: mecanum_flameB:2 ↔ mecanum_polycaplateC:1
- 挿入:205 [Insert]: mecanum_flameB_MIR:2 ↔ mecanum_polycaplateC:1
- 挿入:206 [Insert]: mecanum_flameB:2 ↔ mecanum_polycaplateC:1
- 挿入:207 [Insert]: mecanum_flameB_MIR:2 ↔ mecanum_polycaplateC:1
- 挿入:208 [Insert]: mecanum_flameB_MIR:1 ↔ mecanum_polycaplateC:1
- 挿入:209 [Insert]: mecanum_flameB_MIR:2 ↔ mecanum_polycaplateC:1
- 挿入:210 [Insert]: mecanum_flameB_MIR:1 ↔ mecanum_polycaplateC:1
- 挿入:211 [Insert]: mecanum_flameB:1 ↔ mecanum_polycaplateC:1
- 挿入:212 [Insert]: mecanum_flameB:2 ↔ mecanum_polycaplateC:1
- 挿入:213 [Insert]: mecanum_flameB:2 ↔ mecanum_polycaplateC:1
- 挿入:214 [Insert]: mecanum_flameB:1 ↔ mecanum_polycaplateC:1
- 挿入:215 [Insert]: mecanum_polycaplateA:1 ↔ mecanum_angleA:1
- 挿入:216 [Insert]: mecanum_polycaplateA:1 ↔ mecanum_angleA:1
- 挿入:217 [Insert]: mecanum_polycaplateA:1 ↔ mecanum_angleA:1
- 挿入:218 [Insert]: mecanum_polycaplateA:1 ↔ mecanum_angleA:1
- 挿入:219 [Insert]: mecanum_polycaplate:2 ↔ mecanum_angleA:2
- 挿入:220 [Insert]: mecanum_polycaplate:2 ↔ mecanum_angleA:2
- 挿入:221 [Insert]: mecanum_polycaplate:2 ↔ mecanum_angleA:2
- 挿入:222 [Insert]: mecanum_polycaplate:2 ↔ mecanum_angleA:2
- 挿入:223 [Insert]: mecanum_polycaplateB:1 ↔ mecanum_angleB:1
- 挿入:224 [Insert]: mecanum_polycaplateB:1 ↔ mecanum_angleB:1
- 挿入:225 [Insert]: mecanum_polycaplateB:1 ↔ mecanum_angleB:1
- 挿入:226 [Insert]: mecanum_polycaplateB:1 ↔ mecanum_angleB:1
- 挿入:227 [Insert]: mecanum_polycaplateB:2 ↔ mecanum_angleB:2
- 挿入:228 [Insert]: mecanum_polycaplateB:2 ↔ mecanum_angleB:2
- 挿入:229 [Insert]: mecanum_polycaplateB:2 ↔ mecanum_angleB:2
- 挿入:230 [Insert]: mecanum_polycaplateB:2 ↔ mecanum_angleB:2
- メイト:41 [Mate]: mecanum_shaft:1 ↔ bearingA:1
- メイト:42 [Mate]: motor-wheel_plate:1 ↔ bearingA:1
- 挿入:231 [Insert]: bearingA:1 ↔ mecanum_set_collarA:1
- メイト:43 [Mate]: mecanum_shaft:1 ↔ motor-wheel_plate:2
- 挿入:232 [Insert]: motor-wheel_plate:2 ↔ motor-wheel_plate:3
- 挿入:233 [Insert]: motor-wheel_plate:2 ↔ motor-wheel_plate:3
- 挿入:234 [Insert]: motor-wheel_plate:2 ↔ motor-wheel_plate:3
- 挿入:235 [Insert]: motor-wheel_plate:2 ↔ motor-wheel_plate:3
- 挿入:236 [Insert]: mecanum_flameD:2 ↔ motor-wheel_plate:3
- 挿入:237 [Insert]: mecanum_flameD:2 ↔ motor-wheel_plate:3
- 挿入:238 [Insert]: mecanum_flameD:1 ↔ motor-wheel_plate:3
- 挿入:239 [Insert]: mecanum_flameD:1 ↔ motor-wheel_plate:3
- メイト:44 [Mate]: motor-wheel_plate:2 ↔ bearingA:2
- メイト:45 [Mate]: motor-wheel_plate:2 ↔ bearingA:2
- 挿入:240 [Insert]: bearingA:2 ↔ mecanum_set_collarA:2
- [Insert]: bearingA:3 ↔ mecanum_set_collarA:3
- [Insert]: motor-wheel_plate:4 ↔ motor-wheel_plate:5
- [Insert]: motor-wheel_plate:4 ↔ motor-wheel_plate:5
- [Insert]: motor-wheel_plate:4 ↔ motor-wheel_plate:5
- [Insert]: motor-wheel_plate:4 ↔ motor-wheel_plate:5
- [Mate]: motor-wheel_plate:4 ↔ bearingA:4
- [Mate]: motor-wheel_plate:4 ↔ bearingA:4
- [Insert]: bearingA:4 ↔ mecanum_set_collarA:4
- メイト:48 [Mate]: motor-wheel_plate_MIR:1 ↔ bearingA:3
- メイト:49 [Mate]: mecanum_shaft_MIR:1 ↔ bearingA:3
- メイト:50 [Mate]: mecanum_shaft_MIR:1 ↔ bearingA:4
- 挿入:247 [Insert]: mecanum_flameD:4 ↔ motor-wheel_plate:5
- 挿入:248 [Insert]: mecanum_flameD:4 ↔ motor-wheel_plate:5
- 挿入:249 [Insert]: mecanum_flameD:3 ↔ motor-wheel_plate:5
- 挿入:250 [Insert]: mecanum_flameD:3 ↔ motor-wheel_plate:5
- [Insert]: bearingA:5 ↔ mecanum_set_collarA:5
- [Insert]: motor-wheel_plate:6 ↔ motor-wheel_plate:7
- [Insert]: motor-wheel_plate:6 ↔ motor-wheel_plate:7
- [Insert]: motor-wheel_plate:6 ↔ motor-wheel_plate:7
- [Insert]: motor-wheel_plate:6 ↔ motor-wheel_plate:7
- [Mate]: motor-wheel_plate:6 ↔ bearingA:6
- [Mate]: motor-wheel_plate:6 ↔ bearingA:6
- [Insert]: bearingA:6 ↔ mecanum_set_collarA:6
- [Insert]: bearingA:7 ↔ mecanum_set_collarA:7
- [Insert]: motor-wheel_plate:8 ↔ motor-wheel_plate:9
- [Insert]: motor-wheel_plate:8 ↔ motor-wheel_plate:9
- [Insert]: motor-wheel_plate:8 ↔ motor-wheel_plate:9
- [Insert]: motor-wheel_plate:8 ↔ motor-wheel_plate:9
- [Mate]: motor-wheel_plate:8 ↔ bearingA:8
- [Mate]: motor-wheel_plate:8 ↔ bearingA:8
- [Insert]: bearingA:8 ↔ mecanum_set_collarA:8
- メイト:55 [Mate]: motor-wheel_plate_MIR1:1 ↔ bearingA:5
- メイト:56 [Mate]: mecanum_shaft_MIR1:1 ↔ mecanum_set_collarA:5
- メイト:57 [Mate]: mecanum_shaft_MIR1:1 ↔ bearingA:6
- 挿入:263 [Insert]: mecanum_flameD:2 ↔ motor-wheel_plate:7
- 挿入:264 [Insert]: mecanum_flameD:2 ↔ motor-wheel_plate:7
- 挿入:265 [Insert]: mecanum_flameD:1 ↔ motor-wheel_plate:7
- 挿入:266 [Insert]: mecanum_flameD:1 ↔ motor-wheel_plate:7
- メイト:58 [Mate]: motor-wheel_plate_MIR_MIR:1 ↔ bearingA:7
- メイト:59 [Mate]: mecanum_shaft_MIR_MIR:1 ↔ bearingA:7
- メイト:60 [Mate]: mecanum_shaft_MIR_MIR:1 ↔ bearingA:8
- 挿入:267 [Insert]: mecanum_flameD:3 ↔ motor-wheel_plate:9
- 挿入:268 [Insert]: mecanum_flameD:3 ↔ motor-wheel_plate:9
- 挿入:269 [Insert]: mecanum_flameD:4 ↔ motor-wheel_plate:9
- 挿入:270 [Insert]: mecanum_flameD:4 ↔ motor-wheel_plate:9
- メイト:61 [Mate]: Astuto_enc_wheel:1 ↔ mecanum_encoder_shaftA:1
- メイト:62 [Mate]: mecanum_encoder_shaftA:1 ↔ mecanum_encoder_plateB:1
- メイト:63 [Mate]: Astuto_enc_part1:2 ↔ Astuto_enc_part2:2
- メイト:64 [Mate] (0.2 mm): Astuto_enc_part1:2 ↔ Astuto_enc_part2:2
- 挿入:271 [Insert]: mecanum_encoder_plateB:1 ↔ Astuto_enc_part2:2
- 挿入:272 [Insert]: mecanum_encoder_plateB:1 ↔ Astuto_enc_part2:2
- [Mate]: Astuto_enc_part1:3 ↔ Astuto_enc_part2:3
- 挿入:273 [Insert]: mecanum_encoder_plateB:1 ↔ Astuto_enc_part2:3
- 挿入:274 [Insert]: mecanum_encoder_plateB:1 ↔ Astuto_enc_part2:3
- 挿入:275 [Insert]: mecanum_flameB:4 ↔ Astuto_enc_part1:2
- 挿入:276 [Insert]: mecanum_flameB:4 ↔ Astuto_enc_part1:3
- 挿入:277 [Insert]: mecanum_flameB:1 ↔ Astuto_enc_part1:3
- 挿入:278 [Insert]: mecanum_flameB:1 ↔ Astuto_enc_part1:2
- メイト:66 [Mate] (0.2 mm): Astuto_enc_part1:3 ↔ Astuto_enc_part2:3
- フラッシュ:3 [Flush] (17.307 mm): Astuto_enc_part1:2 ↔ Astuto_enc_part2:2
- メイト:67 [Mate] (3 mm): mecanum_flameB:3 ↔ mecanum_encoder_plateA:1
- メイト:68 [Mate]: mecanum_encoder_shaftA:1 ↔ mecanum_encoder_plateA:1
- 挿入:280 [Insert]: mecanum_encoder_plateB:1 ↔ mecanum_encoder_shaftB:1
- 挿入:281 [Insert]: mecanum_encoder_plateA:1 ↔ mecanum_encoder_shaftB:1
- 挿入:282 [Insert]: mecanum_encoder_plateA:1 ↔ mecanum_encoder_shaftB:2
- 挿入:283 [Insert]: E6A2-CW3C:1 ↔ mecanum_encoder_plateC:1
- 挿入:284 [Insert]: E6A2-CW3C:1 ↔ mecanum_encoder_plateC:1
- メイト:69 [Mate]: mecanum_encoder_shaftA:1 ↔ E6A2-CW3C:1
- フラッシュ:4 [Flush] (6 mm): mecanum_encoder_shaftA:1 ↔ mecanum_encoder_plateA:1
- 挿入:285 [Insert]: mecanum_encoder_plateC:1 ↔ mecanum_encoder_shaftC:1
- 挿入:286 [Insert]: mecanum_encoder_plateC:1 ↔ mecanum_encoder_shaftC:3
- 挿入:287 [Insert]: mecanum_encoder_plateC:1 ↔ mecanum_encoder_shaftC:2
- メイト:70 [Mate]: mecanum_encoder_plateB:1 ↔ mecanum_encoder_shaftC:1
- 挿入:288 [Insert]: mecanum_encoder_plateB:1 ↔ mecanum_encoder_shaftC:3
- 挿入:289 [Insert]: mecanum_encoder_plateB:1 ↔ mecanum_encoder_shaftC:1
- 挿入:290 [Insert]: mecanum_encoder_plateB:1 ↔ mecanum_encoder_shaftC:2
- [Insert]: E6A2-CW3C:2 ↔ mecanum_encoder_plateC:2
- [Insert]: E6A2-CW3C:2 ↔ mecanum_encoder_plateC:2
- 挿入:296 [Insert]: mecanum_flameD:3 ↔ Astuto_enc_part3:1
- 挿入:297 [Insert]: mecanum_flameD:4 ↔ Astuto_enc_part3:1
- 挿入:298 [Insert]: mecanum_flameD:4 ↔ Astuto_enc_part3:2
- 挿入:299 [Insert]: mecanum_flameD:3 ↔ Astuto_enc_part3:2
- メイト:72 [Mate]: Astuto_enc_part3:1 ↔ Astuto_enc_part2:5
- メイト:73 [Mate]: Astuto_enc_part3:2 ↔ Astuto_enc_part2:4
- メイト:74 [Mate] (0.2 mm): Astuto_enc_part3:1 ↔ Astuto_enc_part2:5
- メイト:75 [Mate] (0.2 mm): Astuto_enc_part3:2 ↔ Astuto_enc_part2:4
- 挿入:300 [Insert]: Astuto_enc_part2:4 ↔ mecanum_encoder_plateD:1
- 挿入:301 [Insert]: Astuto_enc_part2:5 ↔ mecanum_encoder_plateD:1
- 挿入:302 [Insert]: Astuto_enc_part2:5 ↔ mecanum_encoder_plateD:1
- 挿入:303 [Insert]: Astuto_enc_part2:4 ↔ mecanum_encoder_plateD:1
- メイト:76 [Mate]: Astuto_enc_wheel:2 ↔ mecanum_encoder_plateD:1